# Autodesk Inventor assembly: Top_Slider Assy
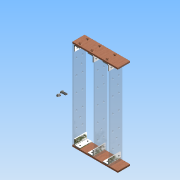
[picture p0: Inventor's stored thumbnail of the model, 180x180]
Saved by Autodesk Inventor 2018.1 (Build 221171000, 171)
## iProperties
Created: 2019-03-18
Part Number: Top_Slider Assy
Document SubType Name: Assembly
Designer: James
Author: James
## Documents named in this file (6)
- C:\Users\admin\Desktop\Ball-Machine\Top Level\Top_Slider Assy.iam
- C:\Users\admin\Desktop\Ball-Machine\Top Level\Top_Slider Piece 1.ipt
- C:\Users\admin\Desktop\Ball-Machine\Top Level\Top_Slider Piece 2.ipt
- C:\Users\admin\Desktop\Ball-Machine\Timing Gate\Timing_Angle Bracket.ipt
- C:\Users\admin\Desktop\Ball-Machine\Timing Gate\Nyloc Nut - M4.ipt
- C:\Users\admin\Desktop\Ball-Machine\Timing Gate\Socket Csk Screw - (A2) - M4 x  16.ipt
## Components (15 placed, 5 different names)
1. Top_Slider Piece 1:1 — Mate:1, Mate:2, Flush:6, Flush:7, Mate:25
2. Top_Slider Piece 2:1 — Flush:1, Flush:2, Flush:3, Mate:1, Flush:4, Flush:5, Flush:6, Mate:3, Mate:4, Mate:11, Mate:12, Mate:13, Mate:14, Mate:15, Mate:16, Mate:17, Mate:18, Mate:19
3. Top_Slider Piece 1:2 — Flush:7, Flush:8, Mate:3, Mate:24
4. Top_Slider Piece 1:3 — Flush:8, Mate:4, Mate:23
5. Top_Slider Piece 2:2 — Mate:2, Flush:4, Flush:5, Mate:5, Mate:6, Mate:7, Flush:9, Flush:10, Mate:8, Mate:9, Mate:10, Mate:20, Mate:21, Mate:22
6. Timing_Angle Bracket:1 — Mate:5, Mate:6, Mate:7, Flush:9, Flush:10, Mate:25
7. Timing_Angle Bracket:2 — Mate:8, Mate:9, Mate:10, Mate:24
8. Timing_Angle Bracket:3 — Mate:11, Mate:12, Mate:13
9. Timing_Angle Bracket:4 — Mate:14, Mate:15, Mate:16
10. Timing_Angle Bracket:5 — Mate:20, Mate:21, Mate:22, Mate:23
11. Timing_Angle Bracket:6 — Mate:17, Mate:18, Mate:19
12. Nyloc Nut - M4:1
13. Socket Csk Screw - (A2) - M4 x  16:1
14. Nyloc Nut - M4:2
15. Socket Csk Screw - (A2) - M4 x  16:2
## Relationships (35: Mate 25, Flush 10)
- Flush:1: Top_Slider Piece 2:1
- Flush:2: Top_Slider Piece 2:1
- Flush:3: Top_Slider Piece 2:1
- Mate:1: Top_Slider Piece 1:1 ↔ Top_Slider Piece 2:1
- Mate:2: Top_Slider Piece 1:1 ↔ Top_Slider Piece 2:2
- Flush:4: Top_Slider Piece 2:1 ↔ Top_Slider Piece 2:2
- Flush:5: Top_Slider Piece 2:1 ↔ Top_Slider Piece 2:2
- Flush:6: Top_Slider Piece 1:1 ↔ Top_Slider Piece 2:1
- Flush:7: Top_Slider Piece 1:1 ↔ Top_Slider Piece 1:2
- Flush:8: Top_Slider Piece 1:2 ↔ Top_Slider Piece 1:3
- Mate:3: Top_Slider Piece 2:1 ↔ Top_Slider Piece 1:2
- Mate:4: Top_Slider Piece 2:1 ↔ Top_Slider Piece 1:3
- Mate:5: Top_Slider Piece 2:2 ↔ Timing_Angle Bracket:1
- Mate:6: Top_Slider Piece 2:2 ↔ Timing_Angle Bracket:1
- Mate:7: Top_Slider Piece 2:2 ↔ Timing_Angle Bracket:1
- Flush:9: Top_Slider Piece 2:2 ↔ Timing_Angle Bracket:1
- Flush:10: Top_Slider Piece 2:2 ↔ Timing_Angle Bracket:1
- Mate:8: Top_Slider Piece 2:2 ↔ Timing_Angle Bracket:2
- Mate:9: Top_Slider Piece 2:2 ↔ Timing_Angle Bracket:2
- Mate:10: Top_Slider Piece 2:2 ↔ Timing_Angle Bracket:2
- Mate:11: Top_Slider Piece 2:1 ↔ Timing_Angle Bracket:3
- Mate:12: Top_Slider Piece 2:1 ↔ Timing_Angle Bracket:3
- Mate:13: Top_Slider Piece 2:1 ↔ Timing_Angle Bracket:3
- Mate:14: Top_Slider Piece 2:1 ↔ Timing_Angle Bracket:4
- Mate:15: Top_Slider Piece 2:1 ↔ Timing_Angle Bracket:4
- Mate:16: Top_Slider Piece 2:1 ↔ Timing_Angle Bracket:4
- Mate:17: Top_Slider Piece 2:1 ↔ Timing_Angle Bracket:6
- Mate:18: Top_Slider Piece 2:1 ↔ Timing_Angle Bracket:6
- Mate:19: Top_Slider Piece 2:1 ↔ Timing_Angle Bracket:6
- Mate:20: Top_Slider Piece 2:2 ↔ Timing_Angle Bracket:5
- Mate:21: Top_Slider Piece 2:2 ↔ Timing_Angle Bracket:5
- Mate:22: Top_Slider Piece 2:2 ↔ Timing_Angle Bracket:5
- Mate:23: Top_Slider Piece 1:3 ↔ Timing_Angle Bracket:5
- Mate:24: Top_Slider Piece 1:2 ↔ Timing_Angle Bracket:2
- Mate:25: Top_Slider Piece 1:1 ↔ Timing_Angle Bracket:1
